# Autodesk Inventor assembly: 揺動節+ヘッケン_MIR
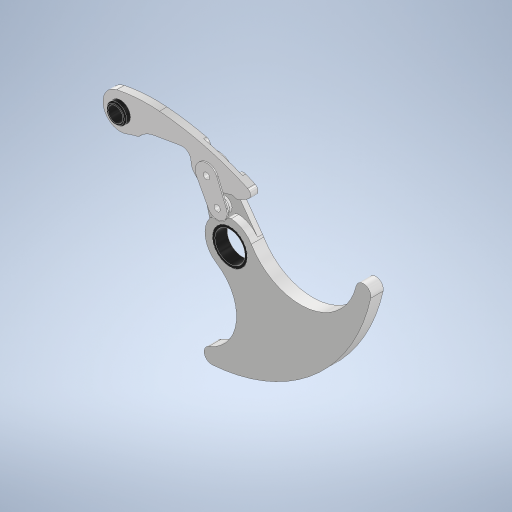
[picture p0: Inventor's stored thumbnail of the model, 512x512]
Saved by Autodesk Inventor 2023 (Build 270158000, 158)
## iProperties
Created: 2022-01-08
Part Number: 揺動節+ヘッケン_MIR
Document SubType Name: Assembly
Designer: muzho
Author: acps
## Documents named in this file (7)
- C:\Users\muzho\Documents\srdc\srdc_2\脚\ミラー\揺動節+ヘッケン_MIR.iam
- C:\Users\muzho\Documents\srdc\srdc_2\脚\ミラー\揺動節_MIR.ipt
- C:\Users\muzho\Documents\srdc\srdc_2\脚\ミラー\ヘッケン_MIR.ipt
- C:\Users\muzho\Documents\srdc\srdc_2\脚\ミラー\ヘッケン抑え_MIR.ipt
- C:\Users\muzho\Documents\srdc\srdc_2\脚\ミラー\w5f12-14n_MIR.ipt
- C:\Users\muzho\Documents\srdc\srdc_2\脚\ミラー\w1.5f5-7n_MIR.ipt
- C:\Users\muzho\Documents\srdc\srdc_2\脚\ミラー\w5f6-12a_MIR.ipt
## Components (6 placed, 6 different names)
1. 揺動節_MIR:1 — 挿入:6, 挿入:5
2. ヘッケン_MIR:1 — 挿入:6, 挿入:8, メイト:2, メイト:1, 挿入:9, 挿入:7
3. ヘッケン抑え_MIR:1 — 挿入:8, メイト:2, メイト:1
4. w5f12-14n_MIR:1 — 挿入:9
5. w1.5f5-7n_MIR:1 — 挿入:7
6. w5f6-12a_MIR:1 — 挿入:5
## Relationships (7: Insert 5, Mate 2)
- 挿入:6 [Insert]: 揺動節_MIR:1 ↔ ヘッケン_MIR:1
- 挿入:8 [Insert]: ヘッケン_MIR:1 ↔ ヘッケン抑え_MIR:1
- メイト:2 [Mate]: ヘッケン_MIR:1 ↔ ヘッケン抑え_MIR:1
- メイト:1 [Mate]: ヘッケン_MIR:1 ↔ ヘッケン抑え_MIR:1
- 挿入:9 [Insert]: ヘッケン_MIR:1 ↔ w5f12-14n_MIR:1
- 挿入:7 [Insert]: ヘッケン_MIR:1 ↔ w1.5f5-7n_MIR:1
- 挿入:5 [Insert]: 揺動節_MIR:1 ↔ w5f6-12a_MIR:1
